# Autodesk Inventor assembly: frame
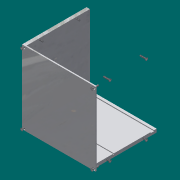
[picture p0: Inventor's stored thumbnail of the model, 180x180]
Saved by Autodesk Inventor 2016 SP2 (Build 200236200, 236)
## iProperties
Created: 2015-10-13
Part Number: frame
Document SubType Name: Assembly
Designer: Sawaiz
Author: Sawaiz
## Documents named in this file (8)
- C:\Users\Sawaiz\oneDrive\projects\modularRICH\frame\frame.iam
- C:\Users\Sawaiz\oneDrive\projects\modularRICH\frame\leftSide.ipt
- C:\Users\Sawaiz\oneDrive\projects\modularRICH\frame\rightSide.ipt
- C:\Users\Sawaiz\oneDrive\projects\modularRICH\frame\bottom.ipt
- C:\Users\Sawaiz\oneDrive\projects\modularRICH\frame\front.ipt
- C:\Users\Sawaiz\oneDrive\projects\modularRICH\frame\top.ipt
- C:\Users\Sawaiz\oneDrive\projects\modularRICH\hardware\4-40x0.5in-flat.ipt
- C:\Users\Sawaiz\oneDrive\projects\modularRICH\modularRICH.xlsx
## Components (17 placed, 6 different names)
1. leftSide:1 — Mate:3, Flush:3, Flush:4, Flush:6, Mate:6, Mate:15, Mate:16, Mate:17, Mate:18, Flush:7, Flush:8, Flush:9, Flush:10
2. rightSide:1 — Flush:1, Mate:2, Flush:4, Mate:4, Flush:5, Mate:7, Mate:8, Mate:9, Mate:10, Flush:15, Flush:16, Flush:17, Flush:18
3. bottom:1 — Flush:1, Mate:1, Flush:2, Mate:2, Mate:3, Flush:3
4. front:1 — Mate:1, Flush:2, Mate:4, Flush:5, Mate:5, Mate:11, Mate:12, Mate:13, Mate:14, Flush:11, Flush:12, Flush:13, Flush:14
5. top:1 — Flush:6, Mate:5, Mate:6
6. 4-40x0.5in-flat:1 — Mate:18, Flush:7
7. 4-40x0.5in-flat:2 — Mate:13, Flush:11
8. 4-40x0.5in-flat:3 — Mate:12, Flush:13
9. 4-40x0.5in-flat:4 — Mate:9, Flush:18
10. 4-40x0.5in-flat:5 — Mate:11, Flush:14
11. 4-40x0.5in-flat:6 — Mate:10, Flush:17
12. 4-40x0.5in-flat:7 — Mate:8, Flush:15
13. 4-40x0.5in-flat:8 — Mate:7, Flush:16
14. 4-40x0.5in-flat:9 — Mate:15, Flush:10
15. 4-40x0.5in-flat:10 — Mate:14, Flush:12
16. 4-40x0.5in-flat:11 — Mate:16, Flush:9
17. 4-40x0.5in-flat:12 — Mate:17, Flush:8
## Relationships (36: Flush 18, Mate 18)
- Flush:1: rightSide:1 ↔ bottom:1
- Mate:1: bottom:1 ↔ front:1
- Flush:2: bottom:1 ↔ front:1
- Mate:2: rightSide:1 ↔ bottom:1
- Mate:3: leftSide:1 ↔ bottom:1
- Flush:3: leftSide:1 ↔ bottom:1
- Flush:4: leftSide:1 ↔ rightSide:1
- Mate:4: rightSide:1 ↔ front:1
- Flush:5: rightSide:1 ↔ front:1
- Flush:6: leftSide:1 ↔ top:1
- Mate:5: front:1 ↔ top:1
- Mate:6: leftSide:1 ↔ top:1
- Mate:7: rightSide:1 ↔ 4-40x0.5in-flat:8
- Mate:8: rightSide:1 ↔ 4-40x0.5in-flat:7
- Mate:9: rightSide:1 ↔ 4-40x0.5in-flat:4
- Mate:10: rightSide:1 ↔ 4-40x0.5in-flat:6
- Mate:11: front:1 ↔ 4-40x0.5in-flat:5
- Mate:12: front:1 ↔ 4-40x0.5in-flat:3
- Mate:13: front:1 ↔ 4-40x0.5in-flat:2
- Mate:14: front:1 ↔ 4-40x0.5in-flat:10
- Mate:15: leftSide:1 ↔ 4-40x0.5in-flat:9
- Mate:16: leftSide:1 ↔ 4-40x0.5in-flat:11
- Mate:17: leftSide:1 ↔ 4-40x0.5in-flat:12
- Mate:18: leftSide:1 ↔ 4-40x0.5in-flat:1
- Flush:7: leftSide:1 ↔ 4-40x0.5in-flat:1
- Flush:8: leftSide:1 ↔ 4-40x0.5in-flat:12
- Flush:9: leftSide:1 ↔ 4-40x0.5in-flat:11
- Flush:10: leftSide:1 ↔ 4-40x0.5in-flat:9
- Flush:11: front:1 ↔ 4-40x0.5in-flat:2
- Flush:12: front:1 ↔ 4-40x0.5in-flat:10
- Flush:13: front:1 ↔ 4-40x0.5in-flat:3
- Flush:14: front:1 ↔ 4-40x0.5in-flat:5
- Flush:15: rightSide:1 ↔ 4-40x0.5in-flat:7
- Flush:16: rightSide:1 ↔ 4-40x0.5in-flat:8
- Flush:17: rightSide:1 ↔ 4-40x0.5in-flat:6
- Flush:18: rightSide:1 ↔ 4-40x0.5in-flat:4
## Named parameters: acrylicThickness = 6.35 mm, aerogelThickness = 30 mm, height = 127 mm, width = 127 mm, depth = 120.142 mm, mirrorAngle = 5 deg, detectorWidth = 52 mm, detectorHeight = 52 mm, mirrorThickness = 3.175 mm, fresnelThickness = 0.254 mm, grooveDensity = 100, focalLength = 76.2 mm, ior = 1.49, centerThickness = 1.27 mm, fresnelAngle = 90 deg, fresnelEffectiveDiameter = 152.4 mm, mirrorSuppourtWidth = 38.1 mm, backGrooveBit = 4.8006 mm, sensorHolderWidth = 88.9 mm, sensorHolderSensorWidth = 53.975 mm, sensorHolderSesnorHeight = 53.975 mm, sensorHolderHeight = 88.9 mm, sensorHolderSensorHeight = 53.975 mm, sensorHolderORingGroove = 3.175 mm, sensorHolderORing = 3.175 mm, sensorHolderFlushORingID = 304.8 mm, sensorHolderFlushORing = 3.175 mm, frontBackORingID = 419.1 mm, oRingWidth = 1.5875 mm, sensorHolderORingID = 203.2 mm, topBottomHorizontalMirrorGroove = 12.7 mm, backMirrorGroove = 6.35 mm, mirrorGroove = 19.05 mm, compressionPercent = 40, fresnelChamfer = 6.35 mm, mirrorGrooveFillet = 6.35 mm, mirrorGrooveDrill = 6.35 mm, mirrorGrooveMill = 3.175 mm, fresnelMirrorChamfer = 6.35 mm, detectorOpeningHeight = 76.2 mm, detectorOpeningWidth = 76.2 mm, sensorHolderDepth = 19.05 mm, frameAcrylicThickness = 9.525 mm, internalAcrylicThicnkess = 6.35 mm, aerogelWidth = 110 mm, aerogelHeight = 110 mm, internalAcrylicThickness = 6.35 mm, aerogelClearence = 3.175 mm, backplanePCBHeight = 76.2 mm, backplaneHoleOffsett = 6.35 mm, backplanePCBWidth = 76.2 mm, backplanePostionOffsett = 12.7 mm, moduleSlotClearence = 0.79375 mm, testMountWidth = 300 mm, testMountHeight = 300 mm, testMountLength = 500 mm, plasticThickness = 6.35 mm, aerogelHolderDepth = 37.30625 mm, caseThickness = 6.35 mm, alignmantGrooveDepth = 1.5875 mm, alignmentGrooveDepth = 1.5875 mm, alignmentGrooveClearance = 0.1016 mm, frontPanelThickness = 2.38125 mm
